# Autodesk Inventor assembly: joint3_as
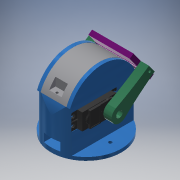
[picture p0: Inventor's stored thumbnail of the model, 180x180]
Saved by Autodesk Inventor 2019 (Build 230136000, 136)
## iProperties
Created: 2019-12-29
Part Number: joint3_as
Material: Типовые
Document SubType Name: Assembly
Designer: Петров Иван
Author: Петров Иван
## Documents named in this file (6)
- E:\IVAN\Ivan_desktop\GitHub\Arm_manip\hardware\joint3_as.iam
- E:\IVAN\Ivan_desktop\GitHub\Arm_manip\hardware\joint3_main.ipt
- E:\IVAN\Ivan_desktop\GitHub\Arm_manip\hardware\Standart_things\tower prone.ipt
- E:\IVAN\Ivan_desktop\GitHub\Arm_manip\hardware\joint3_rot.ipt
- E:\IVAN\Ivan_desktop\GitHub\Arm_manip\hardware\joint3_rot_con.ipt
- E:\IVAN\Ivan_desktop\GitHub\Arm_manip\hardware\joint3_cap.ipt
## Components (6 placed, 5 different names)
1. joint3_main:1 — Совмещение:1, Совмещение:2, Совмещение:3, Совмещение:6, Совмещение:7, Совмещение:12, Совмещение:13, Совмещение:14
2. tower prone:1 — Совмещение:1, Совмещение:2, Совмещение:3, Совмещение:4, Совмещение:5
3. joint3_rot:1 — Совмещение:4, Совмещение:5, Совмещение:9, Совмещение:11, Заподлицо:1
4. joint3_rot:2 — Совмещение:6, Совмещение:7, Совмещение:10
5. joint3_rot_con:1 — Совмещение:9, Совмещение:10, Совмещение:11, Заподлицо:1
6. joint3_cap:1 — Совмещение:12, Совмещение:13, Совмещение:14
## Relationships (14: Mate 13, Flush 1)
- Совмещение:1 [Mate]: joint3_main:1 ↔ tower prone:1
- Совмещение:2 [Mate]: joint3_main:1 ↔ tower prone:1
- Совмещение:3 [Mate]: joint3_main:1 ↔ tower prone:1
- Совмещение:4 [Mate]: tower prone:1 ↔ joint3_rot:1
- Совмещение:5 [Mate]: tower prone:1 ↔ joint3_rot:1
- Совмещение:6 [Mate]: joint3_main:1 ↔ joint3_rot:2
- Совмещение:7 [Mate]: joint3_main:1 ↔ joint3_rot:2
- Совмещение:9 [Mate]: joint3_rot:1 ↔ joint3_rot_con:1
- Совмещение:10 [Mate]: joint3_rot:2 ↔ joint3_rot_con:1
- Совмещение:11 [Mate]: joint3_rot:1 ↔ joint3_rot_con:1
- Заподлицо:1 [Flush]: joint3_rot:1 ↔ joint3_rot_con:1
- Совмещение:12 [Mate]: joint3_main:1 ↔ joint3_cap:1
- Совмещение:13 [Mate]: joint3_main:1 ↔ joint3_cap:1
- Совмещение:14 [Mate]: joint3_main:1 ↔ joint3_cap:1
